# Autodesk Inventor assembly: UpperBody
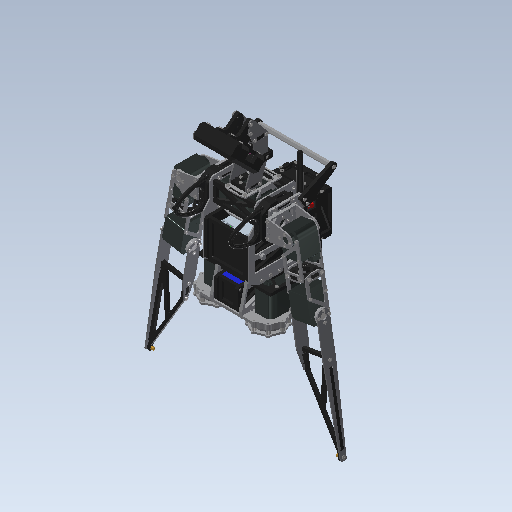
[picture p0: Inventor's stored thumbnail of the model, 512x512]
Saved by Autodesk Inventor 2020.4 (Build 244396010, 396A)
## iProperties
Created: 2016-05-03
Part Number: UpperBody
Document SubType Name: Assembly
Designer: hiroaki
Mass: 2450.59 g
Surface Area: 8110.23 cm^2
Volume: 1381.3 cm^3
Density: 1.77412 g/cm^3
Author: hiroaki
## Documents named in this file (9)
- C:\Users\t-nagamine\Documents\Cit Brains\OpenPlatform_ver3_0\UpperBody\UpperBody.iam
- C:\Users\t-nagamine\Documents\Cit Brains\OpenPlatform_ver3_0\UpperBody\Trunk\Trunk.iam
- C:\Users\t-nagamine\Documents\Cit Brains\OpenPlatform_ver3_0\UpperBody\Head\Head.iam
- C:\Users\t-nagamine\Documents\Cit Brains\OpenPlatform_ver3_0\UpperBody\Arm\ForeArm.iam
- C:\Users\t-nagamine\Documents\Cit Brains\OpenPlatform_ver3_0\UpperBody\Arm\Shoulder.iam
- C:\Users\t-nagamine\Documents\Cit Brains\OpenPlatform_ver3_0\UpperBody\Arm\RightUpperArm.iam
- C:\Users\t-nagamine\Documents\Cit Brains\OpenPlatform_ver3_0\Ready_Made\Screw\M2_6-6.ipt
- C:\Users\t-nagamine\Documents\Cit Brains\OpenPlatform_ver3_0\Ready_Made\Screw\M2_6-8.ipt
- C:\Users\t-nagamine\Documents\Cit Brains\OpenPlatform_ver3_0\UpperBody\Arm\LeftUpperArm.iam
## Components (52 placed, 8 different names)
1. Head:1 [sub-assembly] — 挿入:13, 角度:12, 挿入:82, 挿入:83, 挿入:84, 挿入:85
2. Trunk:1 [sub-assembly] — 挿入:13, 角度:12, 挿入:22, 挿入:23, 角度:22, フラッシュ:10, 角度:25, 角度:26
3. ForeArm:1 [sub-assembly] — 角度:18, 挿入:66, 挿入:67, 挿入:68, 挿入:69, 挿入:70, 挿入:71, 挿入:72, 挿入:73, 挿入:87
4. ForeArm:2 [sub-assembly] — 挿入:19, 角度:18, 挿入:74, 挿入:75, 挿入:76, 挿入:77, 挿入:78, 挿入:79, 挿入:80, 挿入:81
5. RightUpperArm:1 [sub-assembly] — 挿入:19, 挿入:24, 角度:25
6. LeftUpperArm:1 [sub-assembly] — 挿入:86, 角度:26, 挿入:87
7. Shoulder:1 [sub-assembly] — 挿入:22, 角度:22, 角度:23, 挿入:42, 挿入:43, 挿入:44, 挿入:45, 挿入:46, 挿入:47, 挿入:48, 挿入:49, 挿入:50, 挿入:51, 挿入:52, 挿入:53, 挿入:86
8. Shoulder:2 [sub-assembly] — 挿入:23, 挿入:24, 角度:23, 挿入:54, 挿入:55, 挿入:56, 挿入:57, 挿入:58, 挿入:59, 挿入:60, 挿入:61, 挿入:62, 挿入:63, 挿入:64, 挿入:65
9. M2_6-6:1 — 挿入:42
10. M2_6-6:2 — 挿入:43
11. M2_6-6:3 — 挿入:44
12. M2_6-6:4 — 挿入:45
13. M2_6-6:5 — 挿入:46
14. M2_6-6:6 — 挿入:47
15. M2_6-6:7 — 挿入:48
16. M2_6-6:8 — 挿入:49
17. M2_6-6:9 — 挿入:50
18. M2_6-6:10 — 挿入:51
19. M2_6-6:11 — 挿入:52
20. M2_6-6:12 — 挿入:53
21. M2_6-6:13 — 挿入:54
22. M2_6-6:14 — 挿入:55
23. M2_6-6:15 — 挿入:56
24. M2_6-6:16 — 挿入:57
25. M2_6-6:17 — 挿入:58
26. M2_6-6:18 — 挿入:59
27. M2_6-6:19 — 挿入:60
28. M2_6-6:20 — 挿入:61
29. M2_6-6:21 — 挿入:62
30. M2_6-6:22 — 挿入:63
31. M2_6-6:23 — 挿入:64
32. M2_6-6:24 — 挿入:65
33. M2_6-6:25 — 挿入:66
34. M2_6-6:26 — 挿入:67
35. M2_6-6:27 — 挿入:68
36. M2_6-6:28 — 挿入:69
37. M2_6-6:29 — 挿入:70
38. M2_6-6:30 — 挿入:71
39. M2_6-6:31 — 挿入:72
40. M2_6-6:32 — 挿入:73
41. M2_6-6:33 — 挿入:74
42. M2_6-6:34 — 挿入:75
43. M2_6-6:35 — 挿入:76
44. M2_6-6:36 — 挿入:77
45. M2_6-6:37 — 挿入:78
46. M2_6-6:38 — 挿入:79
47. M2_6-6:39 — 挿入:81
48. M2_6-6:40 — 挿入:80
49. M2_6-8:1 — 挿入:82
50. M2_6-8:2 — 挿入:83
51. M2_6-8:3 — 挿入:84
52. M2_6-8:4 — 挿入:85
## Relationships (58: Insert 51, Angle 6, Flush 1)
- 挿入:13 [Insert]: Head:1 ↔ Trunk:1
- 角度:12 [Angle] (0 deg): Head:1 ↔ Trunk:1
- 挿入:19 [Insert]: ForeArm:2 ↔ RightUpperArm:1
- 角度:18 [Angle] (0 deg): ForeArm:1 ↔ ForeArm:2
- 挿入:22 [Insert]: Trunk:1 ↔ Shoulder:1
- 挿入:23 [Insert]: Trunk:1 ↔ Shoulder:2
- 挿入:24 [Insert]: RightUpperArm:1 ↔ Shoulder:2
- 角度:22 [Angle] (0 deg): Trunk:1 ↔ Shoulder:1
- 角度:23 [Angle] (0 deg): Shoulder:1 ↔ Shoulder:2
- 挿入:42 [Insert]: Shoulder:1 ↔ M2_6-6:1
- 挿入:43 [Insert]: Shoulder:1 ↔ M2_6-6:2
- 挿入:44 [Insert]: Shoulder:1 ↔ M2_6-6:3
- 挿入:45 [Insert]: Shoulder:1 ↔ M2_6-6:4
- 挿入:46 [Insert]: Shoulder:1 ↔ M2_6-6:5
- 挿入:47 [Insert]: Shoulder:1 ↔ M2_6-6:6
- 挿入:48 [Insert]: Shoulder:1 ↔ M2_6-6:7
- 挿入:49 [Insert]: Shoulder:1 ↔ M2_6-6:8
- 挿入:50 [Insert]: Shoulder:1 ↔ M2_6-6:9
- 挿入:51 [Insert]: Shoulder:1 ↔ M2_6-6:10
- 挿入:52 [Insert]: Shoulder:1 ↔ M2_6-6:11
- 挿入:53 [Insert]: Shoulder:1 ↔ M2_6-6:12
- 挿入:54 [Insert]: Shoulder:2 ↔ M2_6-6:13
- 挿入:55 [Insert]: Shoulder:2 ↔ M2_6-6:14
- 挿入:56 [Insert]: Shoulder:2 ↔ M2_6-6:15
- 挿入:57 [Insert]: Shoulder:2 ↔ M2_6-6:16
- 挿入:58 [Insert]: Shoulder:2 ↔ M2_6-6:17
- 挿入:59 [Insert]: Shoulder:2 ↔ M2_6-6:18
- 挿入:60 [Insert]: Shoulder:2 ↔ M2_6-6:19
- 挿入:61 [Insert]: Shoulder:2 ↔ M2_6-6:20
- 挿入:62 [Insert]: Shoulder:2 ↔ M2_6-6:21
- 挿入:63 [Insert]: Shoulder:2 ↔ M2_6-6:22
- 挿入:64 [Insert]: Shoulder:2 ↔ M2_6-6:23
- 挿入:65 [Insert]: Shoulder:2 ↔ M2_6-6:24
- 挿入:66 [Insert]: ForeArm:1 ↔ M2_6-6:25
- 挿入:67 [Insert]: ForeArm:1 ↔ M2_6-6:26
- 挿入:68 [Insert]: ForeArm:1 ↔ M2_6-6:27
- 挿入:69 [Insert]: ForeArm:1 ↔ M2_6-6:28
- 挿入:70 [Insert]: ForeArm:1 ↔ M2_6-6:29
- 挿入:71 [Insert]: ForeArm:1 ↔ M2_6-6:30
- 挿入:72 [Insert]: ForeArm:1 ↔ M2_6-6:31
- 挿入:73 [Insert]: ForeArm:1 ↔ M2_6-6:32
- 挿入:74 [Insert]: ForeArm:2 ↔ M2_6-6:33
- 挿入:75 [Insert]: ForeArm:2 ↔ M2_6-6:34
- 挿入:76 [Insert]: ForeArm:2 ↔ M2_6-6:35
- 挿入:77 [Insert]: ForeArm:2 ↔ M2_6-6:36
- 挿入:78 [Insert]: ForeArm:2 ↔ M2_6-6:37
- 挿入:79 [Insert]: ForeArm:2 ↔ M2_6-6:38
- 挿入:80 [Insert]: ForeArm:2 ↔ M2_6-6:40
- 挿入:81 [Insert]: ForeArm:2 ↔ M2_6-6:39
- 挿入:82 [Insert]: Head:1 ↔ M2_6-8:1
- 挿入:83 [Insert]: Head:1 ↔ M2_6-8:2
- 挿入:84 [Insert]: Head:1 ↔ M2_6-8:3
- 挿入:85 [Insert]: Head:1 ↔ M2_6-8:4
- フラッシュ:10 [Flush]: Trunk:1
- 角度:25 [Angle] (10 deg): Trunk:1 ↔ RightUpperArm:1
- 挿入:86 [Insert]: LeftUpperArm:1 ↔ Shoulder:1
- 角度:26 [Angle] (-10 deg): Trunk:1 ↔ LeftUpperArm:1
- 挿入:87 [Insert]: ForeArm:1 ↔ LeftUpperArm:1
